# Autodesk Inventor assembly: front pannel
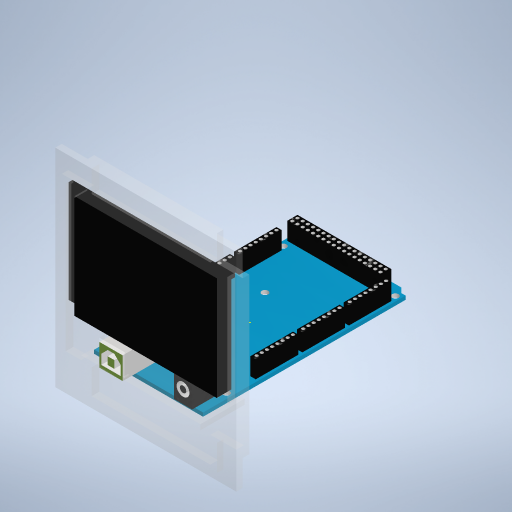
[picture p0: Inventor's stored thumbnail of the model, 512x512]
Saved by Autodesk Inventor 2023 (Build 270158000, 158)
## iProperties
Created: 2023-10-11
Part Number: front pannel
Document SubType Name: Assembly
Designer: Gage
Author: Gage
## Documents named in this file (4)
- C:\Users\Gage\OneDrive\Desktop\Autodesk Inventor\207\front pannel.iam
- C:\Users\Gage\OneDrive\Desktop\Autodesk Inventor\207\FrontPLate.ipt
- C:\Users\Gage\OneDrive\Desktop\Autodesk Inventor\207\Arduino.ipt
- C:\Users\Gage\OneDrive\Desktop\Autodesk Inventor\207\screen.ipt
## Components (3 placed, 3 different names)
1. FrontPLate:1 — Flush:1, Mate:1, Mate:2, Mate:3, Mate:4, Mate:5
2. Arduino:1 — Flush:1, Mate:1, Mate:2
3. screen:1 — Mate:3, Mate:4, Mate:5
## Relationships (6: Mate 5, Flush 1)
- Flush:1: FrontPLate:1 ↔ Arduino:1
- Mate:1: FrontPLate:1 ↔ Arduino:1
- Mate:2: FrontPLate:1 ↔ Arduino:1
- Mate:3: FrontPLate:1 ↔ screen:1
- Mate:4: FrontPLate:1 ↔ screen:1
- Mate:5: FrontPLate:1 ↔ screen:1
